# Autodesk Inventor assembly: Shooter_assembly
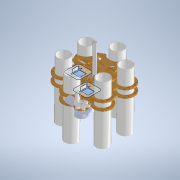
[picture p0: Inventor's stored thumbnail of the model, 180x180]
Saved by Autodesk Inventor 2020.1 (Build 241239000, 239)
## iProperties
Created: 2019-11-06
Part Number: Shooter_assembly
Document SubType Name: Assembly
Designer: Paul Lefeuvre
Mass: 3189.14 g
Surface Area: 13283.7 cm^2
Volume: 3064.78 cm^3
Density: 1.04058 g/cm^3
Author: Paul Lefeuvre
## Documents named in this file (11)
- C:\Users\Paul Lefeuvre\Documents\Inventor\T-Shirt_Cannon\Shooter_assembly.iam
- C:\Users\Paul Lefeuvre\Documents\Inventor\T-Shirt_Cannon\AmmoHolder.ipt
- C:\Users\Paul Lefeuvre\Documents\Inventor\T-Shirt_Cannon\GenevaHolder.ipt
- C:\Users\Paul Lefeuvre\Documents\Inventor\T-Shirt_Cannon\PVC_pipe.ipt
- C:\Users\Paul Lefeuvre\Documents\Inventor\T-Shirt_Cannon\am-2235a Snow Blower Motor With Hex Shaft.ipt
- C:\Users\Paul Lefeuvre\Documents\Inventor\T-Shirt_Cannon\20mm Bearing.ipt
- C:\Users\Paul Lefeuvre\Documents\Inventor\T-Shirt_Cannon\Axle1.ipt
- C:\Users\Paul Lefeuvre\Documents\Inventor\T-Shirt_Cannon\GenevaDrive3.ipt
- C:\Users\Paul Lefeuvre\Documents\Inventor\T-Shirt_Cannon\GenevaDrive2.ipt
- C:\Users\Paul Lefeuvre\Documents\Inventor\T-Shirt_Cannon\GenevaPin.ipt
- C:\Users\Paul Lefeuvre\Documents\Inventor\T-Shirt_Cannon\PVC_connector.ipt
## Components (22 placed, 10 different names)
1. AmmoHolder:1 — Rotational:7, Rigid:21, Rigid:22, Rotational:13, Rotational:14, Rotational:15, Rigid:23
2. GenevaHolder:1 — Rotational:11, Rotational:12
3. PVC_pipe:1 — Rigid:16, Rotational:14
4. PVC_pipe:2 — Rigid:18, Rigid:23
5. PVC_pipe:3 — Rigid:15, Rotational:15
6. PVC_pipe:4 — Rigid:19, Rigid:21, Rotational:11
7. PVC_pipe:5 — Rigid:20, Rigid:22, Rotational:12, Rigid:24
8. PVC_pipe:6 — Rigid:17, Rotational:13, Rigid:25
9. am-2235a Snow Blower Motor With Hex Shaft:1 — Rotational:10
10. AmmoHolder:2 — Rotational:8, Rigid:24, Rigid:25
11. 20mm Bearing:1 — Rotational:7
12. 20mm Bearing:2 — Rotational:8, Rotational:9
13. Axle1:1 — Rotational:9
14. GenevaDrive3:1 — Rigid:13, Rigid:14
15. GenevaDrive2:1 — Rigid:13, Rotational:10
16. GenevaPin:1 — Rigid:14
17. PVC_connector:1 — Rigid:17
18. PVC_connector:2 — Rigid:16
19. PVC_connector:3 — Rigid:15
20. PVC_connector:4 — Rigid:20
21. PVC_connector:5 — Rigid:19
22. PVC_connector:6 — Rigid:18
## Relationships (22: WeldJoint 13, RevoluteJoint 9)
- Rotational:7 [RevoluteJoint]: AmmoHolder:1 ↔ 20mm Bearing:1
- Rotational:8 [RevoluteJoint]: AmmoHolder:2 ↔ 20mm Bearing:2
- Rotational:9 [RevoluteJoint] (0.6 mm): 20mm Bearing:2 ↔ Axle1:1
- Rigid:13 [WeldJoint]: GenevaDrive3:1 ↔ GenevaDrive2:1
- Rotational:10 [RevoluteJoint] (10 mm): am-2235a Snow Blower Motor With Hex Shaft:1 ↔ GenevaDrive2:1
- Rigid:14 [WeldJoint]: GenevaDrive3:1 ↔ GenevaPin:1
- Rigid:15 [WeldJoint]: PVC_pipe:3 ↔ PVC_connector:3
- Rigid:16 [WeldJoint]: PVC_pipe:1 ↔ PVC_connector:2
- Rigid:17 [WeldJoint]: PVC_pipe:6 ↔ PVC_connector:1
- Rigid:18 [WeldJoint]: PVC_pipe:2 ↔ PVC_connector:6
- Rigid:19 [WeldJoint]: PVC_pipe:4 ↔ PVC_connector:5
- Rigid:20 [WeldJoint]: PVC_pipe:5 ↔ PVC_connector:4
- Rigid:21 [WeldJoint] (-88 mm): AmmoHolder:1 ↔ PVC_pipe:4
- Rotational:11 [RevoluteJoint] (-45 mm): GenevaHolder:1 ↔ PVC_pipe:4
- Rigid:22 [WeldJoint] (-88 mm): AmmoHolder:1 ↔ PVC_pipe:5
- Rotational:12 [RevoluteJoint] (-45 mm): GenevaHolder:1 ↔ PVC_pipe:5
- Rotational:13 [RevoluteJoint] (-88 mm): AmmoHolder:1 ↔ PVC_pipe:6
- Rotational:14 [RevoluteJoint] (-88 mm): AmmoHolder:1 ↔ PVC_pipe:1
- Rotational:15 [RevoluteJoint] (-88 mm): AmmoHolder:1 ↔ PVC_pipe:3
- Rigid:23 [WeldJoint] (-88 mm): AmmoHolder:1 ↔ PVC_pipe:2
- Rigid:24 [WeldJoint] (-131 mm): PVC_pipe:5 ↔ AmmoHolder:2
- Rigid:25 [WeldJoint] (-131 mm): PVC_pipe:6 ↔ AmmoHolder:2
## Named parameters: sa_0 = 45000
note: some values were not read from the file. Shown as the stored number, unit unknown: "sa_0".
